# Autodesk Inventor assembly: Airpods
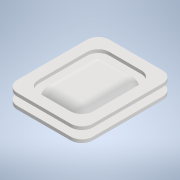
[picture p0: Inventor's stored thumbnail of the model, 180x180]
Saved by Autodesk Inventor 2020 (Build 240168000, 168)
## iProperties
Created: 2020-05-21
Part Number: Airpods
Document SubType Name: Assembly
Designer: maple
Author: maple
## Documents named in this file (3)
- C:\Users\maple\Desktop\Airpods.iam
- C:\Users\maple\Desktop\Airpods Pro Base.ipt
- C:\Users\maple\Desktop\Airpods Pro Top.ipt
## Components (2 placed, 2 different names)
1. Airpods Pro Base:1 — Flush:1, Flush:2
2. Airpods Pro Top:1 — Flush:1, Flush:2
## Relationships (2: Flush 2)
- Flush:1: Airpods Pro Base:1 ↔ Airpods Pro Top:1
- Flush:2: Airpods Pro Base:1 ↔ Airpods Pro Top:1
